# Autodesk Inventor assembly: 8-inch-FIRST-Wheel
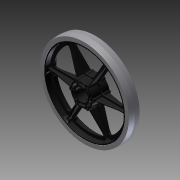
[picture p0: Inventor's stored thumbnail of the model, 180x180]
Saved by Autodesk Inventor 2014 SP1 (Build 180222100, 222)
## iProperties
Created: 2012-01-08
Part Number: 8-inch-FIRST-Wheel
Document SubType Name: Assembly
Designer: Moses
Mass: 366.106 g
Surface Area: 1655.8 cm^2
Volume: 313.358 cm^3
Density: 1.16833 g/cm^3
Translation Standard: STEP AP203
FileName: //Amserv/amserver/AndyMark/Products/Wheels Solid/FIRST Wheel 2010 8 inch/2010 8 wheel.stp
PreProcessor: Unknown
PostProcessor: Build: 190, Release: 2012 SP1 - Date: Mon 08/08/2011
Sent Units: millimeter
Uncertainty: 0.001
Author: Moses
## Documents named in this file (3)
- C:\Users\Moses\Documents\GitHub\frc2014CAD\2012\Repackaged_Team_3061_Yr2012_Ball_Shooter\8-inch-FIRST-Wheel.iam
- C:\Users\Moses\Documents\GitHub\frc2014CAD\2012\Repackaged_Team_3061_Yr2012_Ball_Shooter\8-inch-FIRST-Wheel tread.ipt
- C:\Users\Moses\Documents\GitHub\frc2014CAD\2012\Repackaged_Team_3061_Yr2012_Ball_Shooter\8-inch-FIRST-Wheel hub.ipt
## Components (2 placed, 2 different names)
1. 8-inch-FIRST-Wheel tread:1 — Mate:1, Flush:1
2. 8-inch-FIRST-Wheel hub:1 — Mate:1, Flush:1
## Relationships (2: Mate 1, Flush 1)
- Mate:1: 8-inch-FIRST-Wheel tread:1 ↔ 8-inch-FIRST-Wheel hub:1
- Flush:1: 8-inch-FIRST-Wheel tread:1 ↔ 8-inch-FIRST-Wheel hub:1
